# Autodesk Inventor assembly: Total assembly
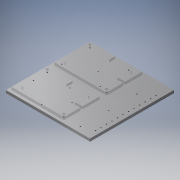
[picture p0: Inventor's stored thumbnail of the model, 180x180]
Saved by Autodesk Inventor 2017 (Build 210142000, 142)
## iProperties
Created: 2016-09-16
Part Number: Total assembly
Document SubType Name: Assembly
Designer: Andreas Fröderberg
Author: Andreas Fröderberg
## Documents named in this file (3)
- C:\Users\Andreas Fröderberg\Documents\Inventor\PCB Fixture\Total assembly.iam
- C:\Users\Andreas Fröderberg\Documents\Inventor\PCB Fixture\Base plate.ipt
- C:\Users\Andreas Fröderberg\Documents\Inventor\PCB Fixture\PCB FIxture 160x100.ipt
## Components (3 placed, 2 different names)
1. Base plate:1 — Mate:1, Mate:2
2. PCB FIxture 160x100:1 — Mate:1
3. PCB FIxture 160x100:2 — Mate:2
## Relationships (2: Mate 2)
- Mate:1: Base plate:1 ↔ PCB FIxture 160x100:1
- Mate:2: Base plate:1 ↔ PCB FIxture 160x100:2
